# Autodesk Inventor assembly: LeadScrewArrangement_MIR
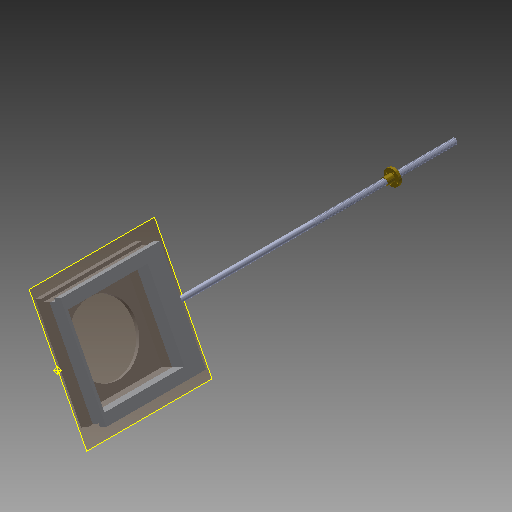
[picture p0: Inventor's stored thumbnail of the model, 512x512]
Saved by Autodesk Inventor 2019 (Build 230136000, 136)
## iProperties
Created: 2019-06-28
Part Number: LeadScrewArrangement_MIR
Document SubType Name: Assembly
Designer: Satwik Pandey
Author: dell
## Documents named in this file (6)
- C:\Users\Satwik Pandey\Desktop\RuTAG Project\New folder\LeadScrewArrangement_MIR.iam
- C:\Users\Satwik Pandey\Desktop\RuTAG Project\New folder\LeadScrewBox_MIR.ipt
- C:\Users\Satwik Pandey\Desktop\RuTAG Project\New folder\LeadScrew_MIR.ipt
- C:\Users\Satwik Pandey\Desktop\RuTAG Project\New folder\LeadScrewNut_MIR.ipt
- C:\Users\Satwik Pandey\Desktop\RuTAG Project\New folder\project flange bearing part1_MIR7_MIR_MIR.ipt
- C:\Users\Satwik Pandey\Desktop\RuTAG Project\New folder\project flange bearing part1_MIR.ipt
## Components (4 placed, 4 different names)
1. LeadScrewBox_MIR:1 — Flush:1, Mate:6
2. LeadScrew_MIR:1 — Mate:7, Mate:6, Mate:8
3. LeadScrewNut_MIR:1 — Mate:8
4. project flange bearing part1_MIR7_MIR_MIR:1
## Relationships (5: Mate 4, Flush 1)
- Flush:1 (-20 mm): LeadScrewBox_MIR:1
- Mate:4
- Mate:7: LeadScrew_MIR:1
- Mate:6: LeadScrewBox_MIR:1 ↔ LeadScrew_MIR:1
- Mate:8: LeadScrew_MIR:1 ↔ LeadScrewNut_MIR:1
